# Autodesk Inventor assembly: maze_version2
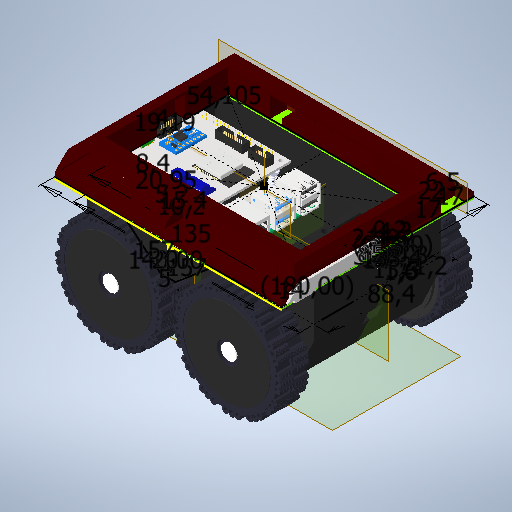
[picture p0: Inventor's stored thumbnail of the model, 512x512]
Saved by Autodesk Inventor 2025 (Build 290162000, 162)
## iProperties
Created: 2026-06-23
Part Number: maze_version2
Document SubType Name: Assembly
Designer: garin
Author: garin
## Documents named in this file (21)
- C:\Users\garin\Documents\Git\TheseusV2_Maze\Construction\Theseus_v2\Theseus_v2.iam
- C:\Users\garin\Documents\Git\TheseusV2_Maze\Construction\Theseus_v2\DDSM210.ipt
- C:\Users\garin\Documents\Git\TheseusV2_Maze\Construction\akkum_TSE\akkum.iam
- C:\Users\garin\Documents\Git\TheseusV2_Maze\Construction\Theseus_v2\low_part.ipt
- C:\Users\garin\Documents\Git\TheseusV2_Maze\Construction\Theseus_v2\USBCamera.ipt
- C:\Users\garin\Documents\Git\TheseusV2_Maze\Construction\maze_test_course\maze_test_course.ipt
- C:\Users\garin\Documents\Git\TheseusV2_Maze\Construction\Theseus_v2\TCS34725.ipt
- C:\Users\garin\Documents\Git\TheseusV2_Maze\Construction\Theseus_v2\optopar.ipt
- C:\Users\garin\Documents\Git\TheseusV2_Maze\Construction\Theseus_v2\magasin.ipt
- C:\Users\garin\Documents\Git\TheseusV2_Maze\Construction\Theseus_v2\LD19_v2.ipt
- C:\Users\garin\Documents\Git\TheseusV2_Maze\Construction\Theseus_v2\mother_board\sensor board.ipt
- C:\Users\garin\Documents\Git\TheseusV2_Maze\Construction\Theseus_v2\VL53l1X.ipt
- C:\Users\garin\Documents\Git\TheseusV2_Maze\Construction\Theseus_v2\VL53l1X\VL53l1X_MIR.ipt
- C:\Users\garin\Documents\Git\TheseusV2_Maze\Construction\Theseus_v2\VL53l1X\VL53l1X_MIR1.ipt
- C:\Users\garin\Documents\Git\TheseusV2_Maze\Construction\Theseus_v2\mother_board\mb_mother_board.iam
- C:\Users\garin\Documents\Git\TheseusV2_Maze\Construction\Theseus_v2\OCS-D008 B.ipt
- C:\Users\garin\Documents\Git\TheseusV2_Maze\Construction\Theseus_v2\up_part.ipt
- C:\Users\garin\Documents\Git\TheseusV2_Maze\Construction\Theseus_v2\SS-5GL switch\SS-5GL switch.ipt
- C:\Users\garin\Documents\Git\TheseusV2_Maze\Construction\Theseus_v2\mother_board\Micro limit switch.ipt
- C:\Users\garin\Documents\Git\TheseusV2_Maze\Construction\Theseus_v2\microswitch_cap.ipt
- C:\Users\garin\Documents\models\altium_models\Micro limit switch_MIR5.ipt
## Components (28 placed, 20 different names)
1. low_part:1 — Заподлицо:1, Заподлицо:2, Заподлицо:3, Совмещение:1, Совмещение:2, Совмещение:3, Совмещение:7, Совмещение:8, Совмещение:9, Совмещение:27, Совмещение:28, Совмещение:29, Совмещение:30, Совмещение:31, Совмещение:32, Совмещение:42, Совмещение:43, Совмещение:44, Совмещение:45, Совмещение:46, Совмещение:47, Совмещение:49, Угол:1, Угол:2, Совмещение:52, Совмещение:53, Совмещение:59, Совмещение:60, Заподлицо:13, Совмещение:62, Совмещение:63, Заподлицо:14, Совмещение:64, Совмещение:65, Совмещение:66, Заподлицо:16, Заподлицо:17, Заподлицо:18, Совмещение:68
2. DDSM210:1 — Совмещение:27, Совмещение:28, Совмещение:29, Заподлицо:19
3. DDSM210:2 — Совмещение:1, Совмещение:2, Совмещение:3
4. DDSM210:3 — Совмещение:30, Совмещение:31, Совмещение:32
5. DDSM210:4 — Совмещение:7, Совмещение:8, Совмещение:9
6. akkum:2 [sub-assembly]
7. maze_test_course:1 — Совмещение:35
8. TCS34725:1 — Совмещение:45, Совмещение:46, Совмещение:47
9. optopar:1 — Совмещение:42, Совмещение:43, Совмещение:44
10. USBCamera:2 — Совмещение:49, Угол:1, Совмещение:68
11. magasin:1 — Совмещение:62, Совмещение:63, Заподлицо:14, Заподлицо:15
12. LD19_v2:1 — Угол:2, Совмещение:52, Совмещение:53, Совмещение:61
13. sensor board:1 — Заподлицо:9, Совмещение:54, Заподлицо:10, Совмещение:55, Заподлицо:11, Совмещение:56, Угол:3, Совмещение:57, Заподлицо:12, Совмещение:58, Совмещение:66, Заподлицо:16, Заподлицо:17, Совмещение:67, Совмещение:75, Заподлицо:20, Совмещение:76
14. VL53l1X:1 — Заподлицо:9, Совмещение:54
15. VL53l1X:2 — Угол:3, Совмещение:57, Заподлицо:12
16. VL53l1X:4 — Заподлицо:11, Совмещение:56, Совмещение:58
17. VL53l1X:5 — Заподлицо:10, Совмещение:55
18. VL53l1X_MIR:1
19. VL53l1X_MIR1:1
20. mb_mother_board:1 [sub-assembly] — Совмещение:59, Совмещение:60, Заподлицо:13, Совмещение:61
21. OCS-D008 B:1 — Заподлицо:15, Совмещение:64, Совмещение:65
22. up_part:1 — Совмещение:67, Заподлицо:18, Заподлицо:19, Совмещение:69, Совмещение:70, Совмещение:71, Совмещение:77, Совмещение:78
23. USBCamera:3 — Совмещение:69, Совмещение:70, Совмещение:71
24. USBCamera:4
25. SS-5GL switch:1
26. Micro limit switch:1 — Совмещение:75, Заподлицо:20, Совмещение:76, Совмещение:79
27. microswitch_cap:1 — Совмещение:77, Совмещение:78, Совмещение:79
28. Micro limit switch_MIR5:1
## Relationships (63: Mate 45, Flush 15, Angle 3)
- Заподлицо:1 [Flush]: low_part:1
- Заподлицо:2 [Flush]: low_part:1
- Заподлицо:3 [Flush]: low_part:1
- Совмещение:1 [Mate]: low_part:1 ↔ DDSM210:2
- Совмещение:2 [Mate]: low_part:1 ↔ DDSM210:2
- Совмещение:3 [Mate]: low_part:1 ↔ DDSM210:2
- Совмещение:7 [Mate]: low_part:1 ↔ DDSM210:4
- Совмещение:8 [Mate]: low_part:1 ↔ DDSM210:4
- Совмещение:9 [Mate]: low_part:1 ↔ DDSM210:4
- Совмещение:27 [Mate]: low_part:1 ↔ DDSM210:1
- Совмещение:28 [Mate]: low_part:1 ↔ DDSM210:1
- Совмещение:29 [Mate]: low_part:1 ↔ DDSM210:1
- Совмещение:30 [Mate]: low_part:1 ↔ DDSM210:3
- Совмещение:31 [Mate]: low_part:1 ↔ DDSM210:3
- Совмещение:32 [Mate]: low_part:1 ↔ DDSM210:3
- Совмещение:35 [Mate]: maze_test_course:1
- Совмещение:42 [Mate]: low_part:1 ↔ optopar:1
- Совмещение:43 [Mate]: low_part:1 ↔ optopar:1
- Совмещение:44 [Mate]: low_part:1 ↔ optopar:1
- Совмещение:45 [Mate]: low_part:1 ↔ TCS34725:1
- Совмещение:46 [Mate]: low_part:1 ↔ TCS34725:1
- Совмещение:47 [Mate]: low_part:1 ↔ TCS34725:1
- Совмещение:49 [Mate]: low_part:1 ↔ USBCamera:2
- Угол:1 [Angle] (0 deg): low_part:1 ↔ USBCamera:2
- Угол:2 [Angle] (180 deg): low_part:1 ↔ LD19_v2:1
- Совмещение:52 [Mate]: low_part:1 ↔ LD19_v2:1
- Совмещение:53 [Mate]: low_part:1 ↔ LD19_v2:1
- Заподлицо:9 [Flush]: sensor board:1 ↔ VL53l1X:1
- Совмещение:54 [Mate]: sensor board:1 ↔ VL53l1X:1
- Заподлицо:10 [Flush]: sensor board:1 ↔ VL53l1X:5
- Совмещение:55 [Mate]: sensor board:1 ↔ VL53l1X:5
- Заподлицо:11 [Flush]: sensor board:1 ↔ VL53l1X:4
- Совмещение:56 [Mate]: sensor board:1 ↔ VL53l1X:4
- Угол:3 [Angle] (0 deg): sensor board:1 ↔ VL53l1X:2
- Совмещение:57 [Mate]: sensor board:1 ↔ VL53l1X:2
- Заподлицо:12 [Flush]: sensor board:1 ↔ VL53l1X:2
- Совмещение:58 [Mate] (5 mm): sensor board:1 ↔ VL53l1X:4
- Совмещение:59 [Mate]: low_part:1 ↔ mb_mother_board:1
- Совмещение:60 [Mate]: low_part:1 ↔ mb_mother_board:1
- Заподлицо:13 [Flush] (4 mm): low_part:1 ↔ mb_mother_board:1
- Совмещение:61 [Mate] (2 mm): LD19_v2:1 ↔ mb_mother_board:1
- Совмещение:62 [Mate] (0.2 mm): low_part:1 ↔ magasin:1
- Совмещение:63 [Mate] (0.2 mm): low_part:1 ↔ magasin:1
- Заподлицо:14 [Flush] (1.4 mm): low_part:1 ↔ magasin:1
- Заподлицо:15 [Flush] (-0.4 mm): magasin:1 ↔ OCS-D008 B:1
- Совмещение:64 [Mate] (0.5 mm): low_part:1 ↔ OCS-D008 B:1
- Совмещение:65 [Mate] (0.5 mm): low_part:1 ↔ OCS-D008 B:1
- Совмещение:66 [Mate]: low_part:1 ↔ sensor board:1
- Заподлицо:16 [Flush]: low_part:1 ↔ sensor board:1
- Заподлицо:17 [Flush]: low_part:1 ↔ sensor board:1
- Совмещение:67 [Mate]: sensor board:1 ↔ up_part:1
- Заподлицо:18 [Flush]: low_part:1 ↔ up_part:1
- Заподлицо:19 [Flush]: DDSM210:1 ↔ up_part:1
- Совмещение:68 [Mate]: low_part:1 ↔ USBCamera:2
- Совмещение:69 [Mate]: up_part:1 ↔ USBCamera:3
- Совмещение:70 [Mate] (0.5 mm): up_part:1 ↔ USBCamera:3
- Совмещение:71 [Mate] (0.5 mm): up_part:1 ↔ USBCamera:3
- Совмещение:75 [Mate]: sensor board:1 ↔ Micro limit switch:1
- Заподлицо:20 [Flush] (2.6 mm): sensor board:1 ↔ Micro limit switch:1
- Совмещение:76 [Mate] (-3 mm): sensor board:1 ↔ Micro limit switch:1
- Совмещение:77 [Mate] (0.25 mm): up_part:1 ↔ microswitch_cap:1
- Совмещение:78 [Mate] (0.2 mm): up_part:1 ↔ microswitch_cap:1
- Совмещение:79 [Mate]: Micro limit switch:1 ↔ microswitch_cap:1
